# Autodesk Inventor assembly: Lever
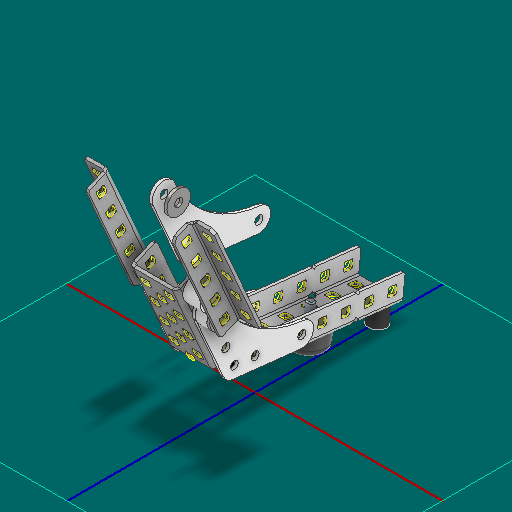
[picture p0: Inventor's stored thumbnail of the model, 512x512]
Saved by Autodesk Inventor 2025 (Build 290162000, 162)
## iProperties
Created: 2024-10-22
Part Number: Lever
Document SubType Name: Assembly
Designer: averey
Author: averey
## Documents named in this file (17)
- C:\Users\avere\VEX\High Stakes\CAD\V2\Clamp\Lever.iam
- C:\Users\avere\VEX\High Stakes\CAD\ROBOPROS-CAD-Inventor\Structure\C Channel\Aluminum 1x2x1\Alu C 1x2x1x5.ipt
- C:\Users\avere\VEX\High Stakes\CAD\V2\Clamp\Custom Parts\60 Degree Gusset.ipt
- C:\Users\avere\VEX\High Stakes\CAD\ROBOPROS-CAD-Inventor\Structure\Standoff\Standoff 1.00.ipt
- C:\Users\avere\VEX\High Stakes\CAD\ROBOPROS-CAD-Inventor\Structure\C Channel\Aluminum 1x2x1\Alu C 1x2x1x4.ipt
- C:\Users\avere\VEX\High Stakes\CAD\ROBOPROS-CAD-Inventor\Structure\C Channel\Aluminum 1x2x1\Alu C 1x2x1x6.ipt
- C:\Users\avere\VEX\High Stakes\CAD\ROBOPROS-CAD-Inventor\Structure\Hardware\Rubber Bumper Smooth.ipt
- D:\VEX\High Stakes\CAD\ROBOPROS-CAD-Inventor\Structure\Standoff.ipt
- C:\Users\avere\VEX\High Stakes\CAD\ROBOPROS-CAD-Inventor\Structure\C Channel\Aluminum 1x2x1\Alu C 1x2x1x7.ipt
- C:\Users\avere\VEX\High Stakes\CAD\ROBOPROS-CAD-Inventor\Motion\Spacers\Spacer Nylon .375 OD\NSpacer .375 OD x .375.ipt
- C:\Users\avere\VEX\High Stakes\CAD\ROBOPROS-CAD-Inventor\Motion\Spacers\Spacer Nylon .375 OD.ipt
- C:\Users\avere\VEX\High Stakes\CAD\ROBOPROS-CAD-Inventor\Structure\Angle\Aluminum 1x1\Alu Angle 1x1x5.ipt
- C:\Users\avere\VEX\High Stakes\CAD\ROBOPROS-CAD-Inventor\Motion\Spacers\Spacer Nylon .500 OD\NSpacer White .500 OD x .250.ipt
- C:\Users\avere\VEX\High Stakes\CAD\ROBOPROS-CAD-Inventor\Motion\Spacers\Spacer Nylon .500 OD.ipt
- C:\Users\avere\VEX\High Stakes\CAD\ROBOPROS-CAD-Inventor\Motion\Spacers\Spacer Nylon .500 OD\NSpacer White .500 OD x .375.ipt
- C:\Users\avere\VEX\High Stakes\CAD\ROBOPROS-CAD-Inventor\Motion\Spacers\Washer Steel\SWasher .500 OD x .062500\SWasher .500 OD x .062500.ipt
- C:\Users\avere\VEX\High Stakes\CAD\ROBOPROS-CAD-Inventor\Motion\Spacers\Washer Steel\SWasher .500 OD x .062500.ipt
## Components (17 placed, 12 different names)
1. Alu C 1x2x1x5:2 — Insert:2, Mate:1, Insert:3, Mate:3, Insert:6, Mate:7
2. 60 Degree Gusset:1 — Insert:2, Mate:1, Mate:5, Insert:5, Mate:6, Insert:26, Insert:28
3. 60 Degree Gusset:2 — Insert:3, Mate:3, Insert:4, Insert:21, Insert:25
4. Standoff 1.00:1 — Insert:4, Mate:5
5. Alu C 1x2x1x4:1 — Insert:5, Mate:6, Mate:9, Mate:10, Insert:27
6. Alu C 1x2x1x6:1 — Insert:6, Mate:7, Mate:8
7. Rubber Bumper Smooth:1 — Insert:24
8. Alu C 1x2x1x7:1 — Insert:21, Mate:8, Insert:22, Insert:23, Insert:24
9. NSpacer .375 OD x .375:1 — Insert:22
10. NSpacer .375 OD x .375:2 — Insert:23
11. Alu Angle 1x1x5:1 — Insert:25, Mate:9
12. Alu Angle 1x1x5:2 — Insert:26, Mate:10
13. NSpacer White .500 OD x .250:1 — Insert:28, Insert:29
14. NSpacer White .500 OD x .375:2 — Insert:27
15. SWasher .500 OD x .062500:1 — Insert:29
16. 60 Degree Gusset:3
17. SWasher .500 OD x .062500:2
## Relationships (22: Insert 14, Mate 8)
- Insert:2: Alu C 1x2x1x5:2 ↔ 60 Degree Gusset:1
- Mate:1: Alu C 1x2x1x5:2 ↔ 60 Degree Gusset:1
- Insert:3: Alu C 1x2x1x5:2 ↔ 60 Degree Gusset:2
- Mate:3: Alu C 1x2x1x5:2 ↔ 60 Degree Gusset:2
- Insert:4: 60 Degree Gusset:2 ↔ Standoff 1.00:1
- Mate:5: 60 Degree Gusset:1 ↔ Standoff 1.00:1
- Insert:5: 60 Degree Gusset:1 ↔ Alu C 1x2x1x4:1
- Mate:6: 60 Degree Gusset:1 ↔ Alu C 1x2x1x4:1
- Insert:6: Alu C 1x2x1x5:2 ↔ Alu C 1x2x1x6:1
- Mate:7: Alu C 1x2x1x5:2 ↔ Alu C 1x2x1x6:1
- Insert:21: 60 Degree Gusset:2 ↔ Alu C 1x2x1x7:1
- Mate:8: Alu C 1x2x1x6:1 ↔ Alu C 1x2x1x7:1
- Insert:22: Alu C 1x2x1x7:1 ↔ NSpacer .375 OD x .375:1
- Insert:23: Alu C 1x2x1x7:1 ↔ NSpacer .375 OD x .375:2
- Insert:24: Rubber Bumper Smooth:1 ↔ Alu C 1x2x1x7:1
- Insert:25 (7.9375 mm): 60 Degree Gusset:2 ↔ Alu Angle 1x1x5:1
- Mate:9: Alu C 1x2x1x4:1 ↔ Alu Angle 1x1x5:1
- Insert:26 (7.9375 mm): 60 Degree Gusset:1 ↔ Alu Angle 1x1x5:2
- Mate:10: Alu C 1x2x1x4:1 ↔ Alu Angle 1x1x5:2
- Insert:27: Alu C 1x2x1x4:1 ↔ NSpacer White .500 OD x .375:2
- Insert:28: 60 Degree Gusset:1 ↔ NSpacer White .500 OD x .250:1
- Insert:29: NSpacer White .500 OD x .250:1 ↔ SWasher .500 OD x .062500:1
